# Autodesk Inventor assembly: Hopper Interface v.2
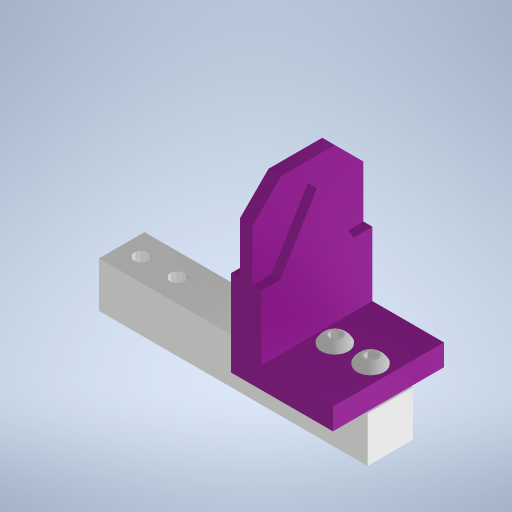
[picture p0: Inventor's stored thumbnail of the model, 512x512]
Saved by Autodesk Inventor 2023 (Build 270158000, 158)
## iProperties
Created: 2022-09-30
Part Number: Hopper Interface v.2
Document SubType Name: Assembly
Designer: Garrett Raker
Author: Garrett Raker
## Documents named in this file (4)
- D:\College Stuff\ATMAE Robotics\Pill Dispenser Robot\Load Cell_Hopper_Connection\Load Cell Hopper Interface Designs\v.2\Hopper Interface v.2.iam
- D:\College Stuff\ATMAE Robotics\Pill Dispenser Robot\Load Cell_Hopper_Connection\Ordered Parts\Load Cell.iam
- D:\College Stuff\ATMAE Robotics\Pill Dispenser Robot\Load Cell_Hopper_Connection\Hopper Connector Designs\v.2\Traingular Hopper Connector v.2.ipt
- D:\College Stuff\ATMAE Robotics\Pill Dispenser Robot\Threads and Fasteners\M4 Button Head Screw 20mm Long.ipt
## Components (4 placed, 3 different names)
1. Load Cell:1 [sub-assembly] — Mate:4, Mate:5, Mate:6, Mate:7
2. Traingular Hopper Connector v.2:1 — Mate:5, Mate:6, Mate:7, Mate:8, Mate:9, Mate:10
3. M4 Button Head Screw 20mm Long:1 — Mate:8, Mate:10
4. M4 Button Head Screw 20mm Long:2 — Mate:4, Mate:9
## Relationships (7: Mate 7)
- Mate:4: Load Cell:1 ↔ M4 Button Head Screw 20mm Long:2
- Mate:5: Load Cell:1 ↔ Traingular Hopper Connector v.2:1
- Mate:6: Load Cell:1 ↔ Traingular Hopper Connector v.2:1
- Mate:7: Load Cell:1 ↔ Traingular Hopper Connector v.2:1
- Mate:8: Traingular Hopper Connector v.2:1 ↔ M4 Button Head Screw 20mm Long:1
- Mate:9: Traingular Hopper Connector v.2:1 ↔ M4 Button Head Screw 20mm Long:2
- Mate:10: Traingular Hopper Connector v.2:1 ↔ M4 Button Head Screw 20mm Long:1
